# Autodesk Inventor assembly: X_CarriageL_V2_1_Short
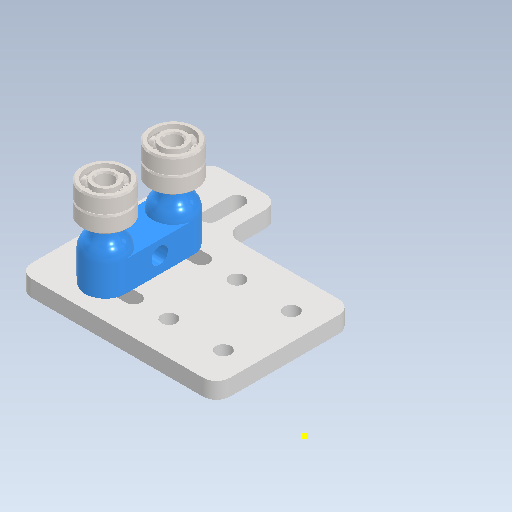
[picture p0: Inventor's stored thumbnail of the model, 512x512]
Saved by Autodesk Inventor 2021 (Build 250183000, 183)
## iProperties
Created: 2021-06-13
Part Number: X_CarriageL_V2_1_Short
Document SubType Name: Assembly
Designer: Jorian Brusind
Author: Jorian Brusind
## Documents named in this file (4)
- C:\Users\Jorian Bruslind\Documents\GitHub\PersonalProjects\HyperRail\Inventor Files\X_CarriageL_V2_1_Short.iam
- C:\Users\Jorian Bruslind\Documents\GitHub\PersonalProjects\HyperRail\Inventor Files\4mm_Roller_Spacer_simple.ipt
- C:\Users\Jorian Bruslind\Documents\GitHub\PersonalProjects\HyperRail\Inventor Files\X_Carriage_Plate_Short.ipt
- C:\Users\Jorian Bruslind\Documents\GitHub\PersonalProjects\HyperRail\Inventor Files\606zz_bearing.ipt
## Components (6 placed, 3 different names)
1. X_Carriage_Plate_Short:1 — Mate:6, Mate:7, Angle:1
2. 4mm_Roller_Spacer_simple:1 — Mate:6, Mate:7, Angle:1, Mate:12, Mate:13, Mate:14
3. 606zz_bearing:1 — Flush:1
4. 606zz_bearing:2 — Mate:12
5. 606zz_bearing:3 — Flush:1, Mate:14
6. 606zz_bearing:4 — Mate:13
## Relationships (11: Mate 9, Angle 1, Flush 1)
- Mate:6: X_Carriage_Plate_Short:1 ↔ 4mm_Roller_Spacer_simple:1
- Mate:7 (-12.5 mm): X_Carriage_Plate_Short:1 ↔ 4mm_Roller_Spacer_simple:1
- Angle:1 (0 deg): X_Carriage_Plate_Short:1 ↔ 4mm_Roller_Spacer_simple:1
- [Mate]: 606zz_bearing:1 ↔ 606zz_bearing:2
- [Mate]: 606zz_bearing:1 ↔ 606zz_bearing:2
- [Mate]: 606zz_bearing:3 ↔ 606zz_bearing:4
- [Mate]: 606zz_bearing:3 ↔ 606zz_bearing:4
- Mate:12: 4mm_Roller_Spacer_simple:1 ↔ 606zz_bearing:2
- Mate:13: 4mm_Roller_Spacer_simple:1 ↔ 606zz_bearing:4
- Flush:1: 606zz_bearing:1 ↔ 606zz_bearing:3
- Mate:14: 4mm_Roller_Spacer_simple:1 ↔ 606zz_bearing:3
## Named parameters: d85_d84 = 0 mm, d87_d86 = 0 mm
